# Autodesk Inventor assembly: Prototype0
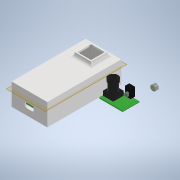
[picture p0: Inventor's stored thumbnail of the model, 180x180]
Saved by Autodesk Inventor 2022 (Build 260153000, 153)
## iProperties
Created: 2022-12-31
Part Number: Prototype0
Document SubType Name: Assembly
Designer: karpova
Author: karpova
## Documents named in this file (11)
- C:\Users\karpova\Desktop\SeniorDesign\24-transcription-study-assistant\cad-files\SeniorDesign_V0\Prototype0.iam
- C:\Users\karpova\Desktop\SeniorDesign\24-transcription-study-assistant\cad-files\SeniorDesign_V0\Camera.ipt
- C:\Users\karpova\Desktop\SeniorDesign\24-transcription-study-assistant\cad-files\SeniorDesign_V0\Driver_Motor.ipt
- C:\Users\karpova\Desktop\SeniorDesign\24-transcription-study-assistant\cad-files\SeniorDesign_V0\MCU_TinyPICO.ipt
- C:\Users\karpova\Desktop\SeniorDesign\24-transcription-study-assistant\cad-files\SeniorDesign_V0\Mic_Omnidirectional.ipt
- C:\Users\karpova\Desktop\SeniorDesign\24-transcription-study-assistant\cad-files\SeniorDesign_V0\Mic_Unidirectional.ipt
- C:\Users\karpova\Desktop\SeniorDesign\24-transcription-study-assistant\cad-files\SeniorDesign_V0\StepperMotor.ipt
- C:\Users\karpova\Desktop\SeniorDesign\24-transcription-study-assistant\cad-files\SeniorDesign_V0\Switch_Base.ipt
- C:\Users\karpova\Desktop\SeniorDesign\24-transcription-study-assistant\cad-files\SeniorDesign_V0\Board_Main.ipt
- C:\Users\karpova\Desktop\SeniorDesign\24-transcription-study-assistant\cad-files\SeniorDesign_V0\Bottom.ipt
- C:\Users\karpova\Desktop\SeniorDesign\24-transcription-study-assistant\cad-files\SeniorDesign_V0\Mid.ipt
## Components (10 placed, 10 different names)
1. Camera:1
2. Driver_Motor:1 — Mate:3, Flush:5
3. MCU_TinyPICO:1 — Flush:4, Mate:2
4. Mic_Omnidirectional:1 — Mate:1
5. Mic_Unidirectional:1
6. StepperMotor:1 — Mate:4, Mate:5, Mate:6, Mate:7, Mate:8
7. Switch_Base:1
8. Board_Main:1 — Mate:1, Flush:1, Flush:2, Flush:3, Flush:4, Mate:2, Mate:3, Flush:5
9. Bottom:1 — Flush:1, Flush:2, Flush:3, Mate:4, Mate:5, Mate:6, Mate:7, Mate:8, Flush:6
10. Mid:1 — Flush:6
## Relationships (14: Mate 8, Flush 6)
- Mate:1: Mic_Omnidirectional:1 ↔ Board_Main:1
- Flush:1: Board_Main:1 ↔ Bottom:1
- Flush:2: Board_Main:1 ↔ Bottom:1
- Flush:3: Board_Main:1 ↔ Bottom:1
- Flush:4: MCU_TinyPICO:1 ↔ Board_Main:1
- Mate:2: MCU_TinyPICO:1 ↔ Board_Main:1
- Mate:3: Driver_Motor:1 ↔ Board_Main:1
- Flush:5: Driver_Motor:1 ↔ Board_Main:1
- Mate:4: StepperMotor:1 ↔ Bottom:1
- Mate:5: StepperMotor:1 ↔ Bottom:1
- Mate:6: StepperMotor:1 ↔ Bottom:1
- Mate:7: StepperMotor:1 ↔ Bottom:1
- Mate:8: StepperMotor:1 ↔ Bottom:1
- Flush:6: Bottom:1 ↔ Mid:1
